# Autodesk Inventor assembly: PowerDistroAssembly_RevB
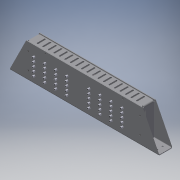
[picture p0: Inventor's stored thumbnail of the model, 180x180]
Saved by Autodesk Inventor 2018 (Build 220112000, 112)
## iProperties
Created: 2018-04-30
Part Number: PowerDistroAssembly_RevB
Document SubType Name: Assembly
Designer: Rich
Author: Rich
## Documents named in this file (8)
- C:\Users\Rich\development\UWaterloo\power-distro.git\SolidModels\PowerDistroAssembly_RevB.iam
- C:\Users\Rich\development\UWaterloo\power-distro.git\SolidModels\Enclosure2_RevB_Outer.ipt
- C:\Users\Rich\development\UWaterloo\power-distro.git\SolidModels\Enclosure2_RevB_Inner.ipt
- C:\Users\Rich\development\UWaterloo\power-distro.git\SolidModels\keystone-PN8425.ipt
- C:\Users\Rich\development\UWaterloo\power-distro.git\SolidModels\6-32x0.25 Slotted Flathead.ipt
- C:\Users\Rich\development\UWaterloo\power-distro.git\SolidModels\power_distro_pcb_RevB.ipt
- C:\Users\Rich\development\UWaterloo\power-distro.git\SolidModels\6-32x0,25 Nut.ipt
- C:\Users\Rich\development\UWaterloo\power-distro.git\SolidModels\rcj-021.iam
## Components (89 placed, 7 different names)
1. Enclosure2_RevB_Outer:1 — Mate:1, Flush:1, Mate:2, Mate:3, Mate:4, Mate:5, Mate:6, Mate:7, Angle:1, Insert:1, Insert:2, Insert:3, Insert:4, Insert:5, Insert:6, Insert:7, Insert:8, Insert:9, Insert:10, Insert:11, Insert:12, Insert:13, Insert:14, Insert:15, Insert:16, Mate:8, Mate:9, Mate:10, Mate:11, Mate:12, Mate:13, Mate:14, Mate:15, Mate:16, Mate:17, Mate:19, Mate:20, Mate:21, Mate:22, Mate:24, Mate:25, Insert:17, Insert:18, Insert:19, Insert:20, Insert:21, Insert:22, Insert:23, Insert:24, Insert:25, Insert:26
2. Enclosure2_RevB_Inner:1 — Mate:3, Mate:4, Mate:5
3. 6-32x0.25 Slotted Flathead:1 — Insert:1
4. 6-32x0.25 Slotted Flathead:2 — Insert:5
5. 6-32x0.25 Slotted Flathead:3 — Insert:3
6. 6-32x0.25 Slotted Flathead:4 — Insert:7
7. 6-32x0.25 Slotted Flathead:5 — Insert:6
8. 6-32x0.25 Slotted Flathead:6 — Insert:2
9. 6-32x0.25 Slotted Flathead:7 — Insert:4
10. 6-32x0.25 Slotted Flathead:8 — Insert:8
11. 6-32x0.25 Slotted Flathead:9 — Insert:11
12. 6-32x0.25 Slotted Flathead:10 — Insert:12, Mate:18
13. 6-32x0.25 Slotted Flathead:11 — Insert:13
14. 6-32x0.25 Slotted Flathead:12 — Insert:10
15. 6-32x0.25 Slotted Flathead:13 — Insert:16
16. 6-32x0.25 Slotted Flathead:14 — Insert:14, Mate:23
17. 6-32x0.25 Slotted Flathead:15 — Insert:9
18. 6-32x0.25 Slotted Flathead:16 — Insert:15
19. keystone-PN8425:1 — Mate:6, Mate:7, Angle:1, Mate:26, Mate:44
20. keystone-PN8425:2 — Mate:11, Mate:19, Mate:40
21. keystone-PN8425:3 — Mate:12, Mate:24, Mate:30
22. keystone-PN8425:4 — Mate:13, Mate:23, Mate:28, Mate:32
23. keystone-PN8425:5 — Mate:14, Mate:22, Mate:51
24. keystone-PN8425:6 — Mate:15, Mate:20, Mate:38
25. keystone-PN8425:7 — Mate:16, Mate:21, Mate:48
26. keystone-PN8425:8 — Mate:10, Mate:25, Mate:27, Mate:34
27. keystone-PN8425:9 — Mate:9, Mate:18, Mate:46
28. keystone-PN8425:10 — Mate:8, Mate:17, Mate:42
29. 6-32x0.25 Slotted Flathead:17 — Insert:17
30. 6-32x0.25 Slotted Flathead:18 — Insert:21
31. 6-32x0.25 Slotted Flathead:19 — Insert:22
32. 6-32x0.25 Slotted Flathead:20 — Insert:20
33. 6-32x0.25 Slotted Flathead:21 — Insert:19
34. 6-32x0.25 Slotted Flathead:22 — Insert:18
35. power_distro_pcb_RevB:1 — Mate:26, Mate:27, Mate:29, Mate:31, Mate:32, Mate:33, Mate:37, Mate:39, Mate:41, Mate:43, Mate:45, Mate:47, Mate:49, Tangent:1, Angle:2, Mate:50
36. 6-32x0,25 Nut:1 — Mate:28, Mate:29
37. 6-32x0,25 Nut:2 — Mate:33, Mate:34
38. 6-32x0,25 Nut:3 — Mate:30, Mate:31
39. 6-32x0,25 Nut:5 — Mate:37, Mate:38
40. 6-32x0,25 Nut:6 — Mate:47, Mate:48
41. 6-32x0,25 Nut:7 — Mate:45, Mate:46
42. 6-32x0,25 Nut:8 — Mate:39, Mate:40
43. 6-32x0,25 Nut:9 — Mate:43, Mate:44
44. 6-32x0,25 Nut:10 — Mate:41, Mate:42
45. 6-32x0.25 Slotted Flathead:23 — Insert:24
46. 6-32x0.25 Slotted Flathead:24 — Insert:23
47. 6-32x0.25 Slotted Flathead:25 — Insert:25
48. 6-32x0.25 Slotted Flathead:26 — Insert:26
49. 6-32x0,25 Nut:11 — Mate:50, Mate:51
50. rcj-021:1 [sub-assembly] — Mate:49, Tangent:1, Angle:2
51. rcj-021:2 [sub-assembly]
52. rcj-021:3 [sub-assembly]
53. rcj-021:4 [sub-assembly]
54. rcj-021:5 [sub-assembly]
55. rcj-021:6 [sub-assembly]
56. rcj-021:7 [sub-assembly]
57. rcj-021:8 [sub-assembly]
58. rcj-021:9 [sub-assembly]
59. rcj-021:10 [sub-assembly]
60. rcj-021:11 [sub-assembly]
61. rcj-021:12 [sub-assembly]
62. rcj-021:13 [sub-assembly]
63. rcj-021:14 [sub-assembly]
64. rcj-021:15 [sub-assembly]
65. rcj-021:16 [sub-assembly]
66. rcj-021:17 [sub-assembly]
67. rcj-021:18 [sub-assembly]
68. rcj-021:19 [sub-assembly]
69. rcj-021:20 [sub-assembly]
70. rcj-021:21 [sub-assembly]
71. rcj-021:22 [sub-assembly]
72. rcj-021:23 [sub-assembly]
73. rcj-021:24 [sub-assembly]
74. rcj-021:25 [sub-assembly]
75. rcj-021:26 [sub-assembly]
76. rcj-021:27 [sub-assembly]
77. rcj-021:28 [sub-assembly]
78. rcj-021:29 [sub-assembly]
79. rcj-021:30 [sub-assembly]
80. rcj-021:31 [sub-assembly]
81. rcj-021:32 [sub-assembly]
82. rcj-021:33 [sub-assembly]
83. rcj-021:34 [sub-assembly]
84. rcj-021:35 [sub-assembly]
85. rcj-021:36 [sub-assembly]
86. rcj-021:37 [sub-assembly]
87. rcj-021:38 [sub-assembly]
88. rcj-021:39 [sub-assembly]
89. rcj-021:40 [sub-assembly]
## Component patterns: (20 elements), (2 elements, first: rcj-021:1), Component Pattern 3:2 (2 elements), Component Pattern 3:3 (2 elements), Component Pattern 3:4 (2 elements), Component Pattern 3:5 (2 elements), Component Pattern 3:6 (2 elements), Component Pattern 3:7 (2 elements), Component Pattern 3:8 (2 elements), Component Pattern 3:9 (2 elements), Component Pattern 3:10 (2 elements), Component Pattern 3:11 (2 elements), Component Pattern 3:12 (2 elements), Component Pattern 3:13 (2 elements), Component Pattern 3:14 (2 elements), Component Pattern 3:15 (2 elements), Component Pattern 3:16 (2 elements), Component Pattern 3:17 (2 elements), Component Pattern 3:18 (2 elements), Component Pattern 3:19 (2 elements), Component Pattern 3:20 (2 elements)
## Relationships (79: Mate 49, Insert 26, Angle 2, Flush 1, Tangent 1)
- Mate:1: Enclosure2_RevB_Outer:1
- Flush:1: Enclosure2_RevB_Outer:1
- Mate:2: Enclosure2_RevB_Outer:1
- Mate:3: Enclosure2_RevB_Outer:1 ↔ Enclosure2_RevB_Inner:1
- Mate:4: Enclosure2_RevB_Outer:1 ↔ Enclosure2_RevB_Inner:1
- Mate:5: Enclosure2_RevB_Outer:1 ↔ Enclosure2_RevB_Inner:1
- Mate:6: Enclosure2_RevB_Outer:1 ↔ keystone-PN8425:1
- Mate:7: Enclosure2_RevB_Outer:1 ↔ keystone-PN8425:1
- Angle:1 (0 deg): Enclosure2_RevB_Outer:1 ↔ keystone-PN8425:1
- Insert:1: Enclosure2_RevB_Outer:1 ↔ 6-32x0.25 Slotted Flathead:1
- Insert:2: Enclosure2_RevB_Outer:1 ↔ 6-32x0.25 Slotted Flathead:6
- Insert:3: Enclosure2_RevB_Outer:1 ↔ 6-32x0.25 Slotted Flathead:3
- Insert:4: Enclosure2_RevB_Outer:1 ↔ 6-32x0.25 Slotted Flathead:7
- Insert:5: Enclosure2_RevB_Outer:1 ↔ 6-32x0.25 Slotted Flathead:2
- Insert:6: Enclosure2_RevB_Outer:1 ↔ 6-32x0.25 Slotted Flathead:5
- Insert:7: Enclosure2_RevB_Outer:1 ↔ 6-32x0.25 Slotted Flathead:4
- Insert:8: Enclosure2_RevB_Outer:1 ↔ 6-32x0.25 Slotted Flathead:8
- Insert:9: Enclosure2_RevB_Outer:1 ↔ 6-32x0.25 Slotted Flathead:15
- Insert:10: Enclosure2_RevB_Outer:1 ↔ 6-32x0.25 Slotted Flathead:12
- Insert:11: Enclosure2_RevB_Outer:1 ↔ 6-32x0.25 Slotted Flathead:9
- Insert:12: Enclosure2_RevB_Outer:1 ↔ 6-32x0.25 Slotted Flathead:10
- Insert:13: Enclosure2_RevB_Outer:1 ↔ 6-32x0.25 Slotted Flathead:11
- Insert:14: Enclosure2_RevB_Outer:1 ↔ 6-32x0.25 Slotted Flathead:14
- Insert:15: Enclosure2_RevB_Outer:1 ↔ 6-32x0.25 Slotted Flathead:16
- Insert:16: Enclosure2_RevB_Outer:1 ↔ 6-32x0.25 Slotted Flathead:13
- Mate:8: Enclosure2_RevB_Outer:1 ↔ keystone-PN8425:10
- Mate:9: Enclosure2_RevB_Outer:1 ↔ keystone-PN8425:9
- Mate:10: Enclosure2_RevB_Outer:1 ↔ keystone-PN8425:8
- Mate:11: Enclosure2_RevB_Outer:1 ↔ keystone-PN8425:2
- Mate:12: Enclosure2_RevB_Outer:1 ↔ keystone-PN8425:3
- Mate:13: Enclosure2_RevB_Outer:1 ↔ keystone-PN8425:4
- Mate:14: Enclosure2_RevB_Outer:1 ↔ keystone-PN8425:5
- Mate:15: Enclosure2_RevB_Outer:1 ↔ keystone-PN8425:6
- Mate:16: Enclosure2_RevB_Outer:1 ↔ keystone-PN8425:7
- Mate:17: Enclosure2_RevB_Outer:1 ↔ keystone-PN8425:10
- Mate:18: 6-32x0.25 Slotted Flathead:10 ↔ keystone-PN8425:9
- Mate:19: Enclosure2_RevB_Outer:1 ↔ keystone-PN8425:2
- Mate:20: Enclosure2_RevB_Outer:1 ↔ keystone-PN8425:6
- Mate:21: Enclosure2_RevB_Outer:1 ↔ keystone-PN8425:7
- Mate:22: Enclosure2_RevB_Outer:1 ↔ keystone-PN8425:5
- Mate:23: 6-32x0.25 Slotted Flathead:14 ↔ keystone-PN8425:4
- Mate:24: Enclosure2_RevB_Outer:1 ↔ keystone-PN8425:3
- Mate:25: Enclosure2_RevB_Outer:1 ↔ keystone-PN8425:8
- Insert:17: Enclosure2_RevB_Outer:1 ↔ 6-32x0.25 Slotted Flathead:17
- Insert:18: Enclosure2_RevB_Outer:1 ↔ 6-32x0.25 Slotted Flathead:22
- Insert:19: Enclosure2_RevB_Outer:1 ↔ 6-32x0.25 Slotted Flathead:21
- Insert:20: Enclosure2_RevB_Outer:1 ↔ 6-32x0.25 Slotted Flathead:20
- Insert:21: Enclosure2_RevB_Outer:1 ↔ 6-32x0.25 Slotted Flathead:18
- Insert:22: Enclosure2_RevB_Outer:1 ↔ 6-32x0.25 Slotted Flathead:19
- Mate:26: keystone-PN8425:1 ↔ power_distro_pcb_RevB:1
- Mate:27: keystone-PN8425:8 ↔ power_distro_pcb_RevB:1
- Mate:28: keystone-PN8425:4 ↔ 6-32x0,25 Nut:1
- Mate:29: power_distro_pcb_RevB:1 ↔ 6-32x0,25 Nut:1
- Mate:30: keystone-PN8425:3 ↔ 6-32x0,25 Nut:3
- Mate:31: power_distro_pcb_RevB:1 ↔ 6-32x0,25 Nut:3
- Mate:32: keystone-PN8425:4 ↔ power_distro_pcb_RevB:1
- Mate:33: power_distro_pcb_RevB:1 ↔ 6-32x0,25 Nut:2
- Mate:34: keystone-PN8425:8 ↔ 6-32x0,25 Nut:2
- Mate:37: power_distro_pcb_RevB:1 ↔ 6-32x0,25 Nut:5
- Mate:38: keystone-PN8425:6 ↔ 6-32x0,25 Nut:5
- Mate:39: power_distro_pcb_RevB:1 ↔ 6-32x0,25 Nut:8
- Mate:40: keystone-PN8425:2 ↔ 6-32x0,25 Nut:8
- Mate:41: power_distro_pcb_RevB:1 ↔ 6-32x0,25 Nut:10
- Mate:42: keystone-PN8425:10 ↔ 6-32x0,25 Nut:10
- Mate:43: power_distro_pcb_RevB:1 ↔ 6-32x0,25 Nut:9
- Mate:44: keystone-PN8425:1 ↔ 6-32x0,25 Nut:9
- Mate:45: power_distro_pcb_RevB:1 ↔ 6-32x0,25 Nut:7
- Mate:46: keystone-PN8425:9 ↔ 6-32x0,25 Nut:7
- Mate:47: power_distro_pcb_RevB:1 ↔ 6-32x0,25 Nut:6
- Mate:48: keystone-PN8425:7 ↔ 6-32x0,25 Nut:6
- Insert:23: Enclosure2_RevB_Outer:1 ↔ 6-32x0.25 Slotted Flathead:24
- Insert:24: Enclosure2_RevB_Outer:1 ↔ 6-32x0.25 Slotted Flathead:23
- Insert:25: Enclosure2_RevB_Outer:1 ↔ 6-32x0.25 Slotted Flathead:25
- Insert:26: Enclosure2_RevB_Outer:1 ↔ 6-32x0.25 Slotted Flathead:26
- Mate:49: power_distro_pcb_RevB:1 ↔ rcj-021:1
- Tangent:1: power_distro_pcb_RevB:1 ↔ rcj-021:1
- Angle:2 (0 deg): power_distro_pcb_RevB:1 ↔ rcj-021:1
- Mate:50: power_distro_pcb_RevB:1 ↔ 6-32x0,25 Nut:11
- Mate:51: keystone-PN8425:5 ↔ 6-32x0,25 Nut:11
